# Autodesk Inventor assembly: 2018 Robot
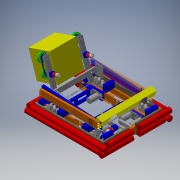
[picture p0: Inventor's stored thumbnail of the model, 180x180]
Saved by Autodesk Inventor 2018 (Build 220112000, 112)
## iProperties
Created: 2018-01-18
Part Number: 2018 Robot
Document SubType Name: Assembly
Designer: Apple
Author: Apple
## Documents named in this file (9)
- C:\Users\Apple\Documents\Inventor\2018 PowerUp\2018 Robot.iam
- C:\Users\Apple\Documents\Inventor\2018 PowerUp\2016 Chassie with 2018 Gearbox.iam
- C:\Users\Apple\Documents\Inventor\2018 PowerUp\Scissor Anchor.ipt
- C:\Users\Apple\Documents\Inventor\2018 PowerUp\2018 Scissor\2018 Scissor.iam
- C:\Users\Apple\Documents\Inventor\2018 PowerUp\2018 Scissor\2018 Scissor Right.iam
- C:\Users\Apple\Documents\Inventor\2018 PowerUp\Cube Intake\Intake 3.iam
- C:\Users\Apple\Documents\Inventor\2018 PowerUp\Cube Intake\2018 Intake Plate.ipt
- C:\Users\Apple\Documents\Inventor\2018 PowerUp\Cube Intake\8in Cyl.iam
- C:\Users\Apple\Documents\Inventor\2018 PowerUp\Hook\Hook Assemly Concept.iam
## Components (10 placed, 8 different names)
1. 2016 Chassie with 2018 Gearbox:3 [sub-assembly] — Mate:1, Flush:1, Flush:2, Mate:14, Flush:5
2. Scissor Anchor:1 — Mate:1, Flush:1, Flush:2, Rotational:1, Flush:3, Flush:4
3. Scissor Anchor:2 — Flush:3, Flush:4, Flush:5, Rotational:2
4. 2018 Scissor Left:1 [sub-assembly] — Rotational:1, Mate:14, Mate:15, Mate:22, Flush:8, Mate:23, Angle:1, Mate:24
5. 2018 Scissor Right:1 [sub-assembly] — Rotational:2, Mate:15, Flush:6, Flush:7, Mate:17, Mate:19, Flush:10
6. Intake 3:1 [sub-assembly] — Mate:18, Mate:19, Angle:1, Mate:25
7. 2018 Intake Plate:1 — Flush:6, Flush:7, Mate:17, Mate:18
8. 2018 Intake Plate:2 — Mate:22, Flush:8, Mate:23
9. 8in Cyl:1 [sub-assembly] — Mate:24, Mate:25
10. Hook Assemly Concept:1 [sub-assembly] — Flush:10
## Relationships (24: Mate 10, Flush 10, RevoluteJoint 3, Angle 1)
- Mate:1 (76.2 mm): 2016 Chassie with 2018 Gearbox:3 ↔ Scissor Anchor:1
- Flush:1 (63.5 mm): 2016 Chassie with 2018 Gearbox:3 ↔ Scissor Anchor:1
- Flush:2 (12.7 mm): 2016 Chassie with 2018 Gearbox:3 ↔ Scissor Anchor:1
- Rotational:1 [RevoluteJoint]: Scissor Anchor:1 ↔ 2018 Scissor Left:1
- Mate:14 (30.099 mm): 2016 Chassie with 2018 Gearbox:3 ↔ 2018 Scissor Left:1
- Flush:3: Scissor Anchor:1 ↔ Scissor Anchor:2
- Flush:4: Scissor Anchor:1 ↔ Scissor Anchor:2
- Flush:5 (12.7 mm): 2016 Chassie with 2018 Gearbox:3 ↔ Scissor Anchor:2
- Rotational:2 [RevoluteJoint]: Scissor Anchor:2 ↔ 2018 Scissor Right:1
- Mate:15: 2018 Scissor Left:1 ↔ 2018 Scissor Right:1
- Flush:6: 2018 Scissor Right:1 ↔ 2018 Intake Plate:1
- Flush:7: 2018 Scissor Right:1 ↔ 2018 Intake Plate:1
- Mate:17: 2018 Scissor Right:1 ↔ 2018 Intake Plate:1
- Mate:18: Intake 3:1 ↔ 2018 Intake Plate:1
- Mate:19 (12.7 mm): 2018 Scissor Right:1 ↔ Intake 3:1
- Mate:22: 2018 Scissor Left:1 ↔ 2018 Intake Plate:2
- Flush:8: 2018 Scissor Left:1 ↔ 2018 Intake Plate:2
- Mate:23 (0.5334 mm): 2018 Scissor Left:1 ↔ 2018 Intake Plate:2
- Angle:1 (-90 deg): 2018 Scissor Left:1 ↔ Intake 3:1
- Mate:24: 2018 Scissor Left:1 ↔ 8in Cyl:1
- Mate:25: Intake 3:1 ↔ 8in Cyl:1
- [Flush]: 2018 Scissor Left:1 ↔ Hook Assemly Concept:1
- [RevoluteJoint]: 2018 Scissor Right:1 ↔ Hook Assemly Concept:1
- Flush:10: 2018 Scissor Right:1 ↔ Hook Assemly Concept:1
